# Autodesk Inventor assembly: Assembly2
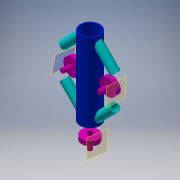
[picture p0: Inventor's stored thumbnail of the model, 180x180]
Saved by Autodesk Inventor 2016 (Build 200138000, 138)
## iProperties
Created: 2017-09-28
Part Number: Assembly2
Document SubType Name: Assembly
Designer: Student
Author: Student
## Documents named in this file (4)
- C:\Users\Student\Documents\Derek Code and Projects\ROV V2\Assembly2.iam
- C:\Users\Student\Documents\Derek Code and Projects\ROV V2\Angled Pipe (Attached to Control Pipe).ipt
- C:\Users\Student\Documents\Derek Code and Projects\ROV V2\Control Pipe V2.ipt
- C:\Users\Student\Documents\Derek Code and Projects\CodeBenderCode-master\ROV CAD Electronics\T100 rough draft.ipt
## Components (8 placed, 3 different names)
1. Angled Pipe (Attached to Control Pipe):3 — Mate:2
2. Angled Pipe (Attached to Control Pipe):4 — Mate:1
3. Control Pipe V2:1 — Mate:1, Mate:2, Mate:3, Mate:4, Mate:5
4. Angled Pipe (Attached to Control Pipe):5 — Mate:4
5. Angled Pipe (Attached to Control Pipe):6 — Mate:3
6. T100 rough draft:2
7. T100 rough draft:3
8. T100 rough draft:4 — Mate:5
## Relationships (5: Mate 5)
- Mate:1: Angled Pipe (Attached to Control Pipe):4 ↔ Control Pipe V2:1
- Mate:2: Angled Pipe (Attached to Control Pipe):3 ↔ Control Pipe V2:1
- Mate:3: Control Pipe V2:1 ↔ Angled Pipe (Attached to Control Pipe):6
- Mate:4: Control Pipe V2:1 ↔ Angled Pipe (Attached to Control Pipe):5
- Mate:5: Control Pipe V2:1 ↔ T100 rough draft:4
